# Autodesk Inventor assembly: ForeArm
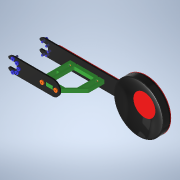
[picture p0: Inventor's stored thumbnail of the model, 180x180]
Saved by Autodesk Inventor 2020 (Build 240168000, 168)
## iProperties
Created: 2022-01-10
Part Number: ForeArm
Document SubType Name: Assembly
Designer: Masato Kubotera
Author: Masato Kubotera
## Documents named in this file (12)
- C:\Users\MasatoKubotera\Documents\Inventor\OpenPlatform_ver3_0 - prototype\UpperBody\Arm\ForeArm.iam
- C:\Users\MasatoKubotera\Documents\Inventor\OpenPlatform_ver3_0 - prototype\UpperBody\Arm\ForeArm_outside_frame.ipt
- C:\Users\MasatoKubotera\Documents\Inventor\OpenPlatform_ver3_0 - prototype\UpperBody\Arm\ForeArm_hand.ipt
- C:\Users\MasatoKubotera\Documents\Inventor\OpenPlatform_ver3_0 - prototype\UpperBody\Arm\ForeArm_inside_frame.ipt
- C:\Users\MasatoKubotera\Documents\Inventor\OpenPlatform_ver3_0 - prototype\ReadyMade\InsertNut\UD-43040.ipt
- C:\Users\MasatoKubotera\Documents\Inventor\OpenPlatform_ver3_0 - prototype\ReadyMade\Screw\M3-6.ipt
- C:\Users\MasatoKubotera\Documents\Inventor\OpenPlatform_ver3_0 - prototype\ReadyMade\Screw\M2_6-6.ipt
- C:\Users\MasatoKubotera\Documents\Inventor\OpenPlatform_ver3_0 - prototype\ReadyMade\InsertNut\IRU-304SW.ipt
- C:\Users\MasatoKubotera\Documents\Inventor\OpenPlatform_ver3_0 - prototype\UpperBody\Arm\ForeArm_diagonal.ipt
- C:\Users\MasatoKubotera\Documents\Inventor\OpenPlatform_ver3_0 - prototype\UpperBody\Arm\ForeArm_outside_cloth.ipt
- C:\Users\MasatoKubotera\Documents\Inventor\OpenPlatform_ver3_0 - prototype\ReadyMade\Bush\L3040-8110TB.ipt
- C:\Users\MasatoKubotera\Documents\Inventor\OpenPlatform_ver3_0 - prototype\ReadyMade\Screw\M3-8.ipt
## Components (34 placed, 11 different names)
1. ForeArm_outside_frame:1 — 挿入:7, 挿入:9, 挿入:10, 挿入:16, 挿入:17, 挿入:23, 挿入:24, 挿入:28, 挿入:31, 挿入:32, 挿入:33, 挿入:34, メイト:1, メイト:2, フラッシュ:1, 挿入:8, 挿入:39, 挿入:41, 挿入:42, 挿入:43
2. ForeArm_hand:1 — 挿入:1, 挿入:2, 挿入:3, 挿入:4, 挿入:8
3. ForeArm_inside_frame:1 — 挿入:25, 挿入:26, 挿入:29, 挿入:30, 挿入:35, 挿入:36, 挿入:37, 挿入:38, 挿入:40
4. ForeArm_diagonal:1 — 挿入:19, 挿入:20, 挿入:21, 挿入:22
5. M2_6-6:9 — 挿入:39
6. M2_6-6:10 — 挿入:40
7. ForeArm_outside_cloth:1 — 挿入:47, 挿入:48, 挿入:49
8. L3040-8110TB:1 — 挿入:41, 挿入:47, 挿入:50
9. L3040-8110TB:2 — 挿入:42, 挿入:48, 挿入:51
10. L3040-8110TB:3 — 挿入:43, 挿入:46, 挿入:49
11. M3-8:2 — 挿入:50
12. M3-8:3 — 挿入:51
13. M3-6:10 — 挿入:30
14. M3-6:9 — 挿入:29
15. M3-6:8 — 挿入:28
16. M2_6-6:8 — 挿入:38
17. M2_6-6:7 — 挿入:37
18. M2_6-6:6 — 挿入:36
19. M2_6-6:5 — 挿入:35
20. M2_6-6:4 — 挿入:34
21. M2_6-6:3 — 挿入:33
22. M2_6-6:2 — 挿入:32
23. M2_6-6:1 — 挿入:31
24. M3-6:5 — 挿入:17
25. M3-6:4 — 挿入:16
26. M3-8:1 — 挿入:46
27. UD-43040:4 — 挿入:4, 挿入:10
28. UD-43040:3 — 挿入:3, 挿入:9
29. UD-43040:2 — 挿入:2
30. UD-43040:1 — 挿入:1, 挿入:7
31. IRU-304SW:1 — 挿入:19, 挿入:23
32. IRU-304SW:2 — 挿入:20, 挿入:24
33. IRU-304SW:3 — 挿入:21, 挿入:25
34. IRU-304SW:4 — 挿入:22, 挿入:26
## Relationships (43: Insert 40, Mate 2, Flush 1)
- 挿入:1 [Insert]: ForeArm_hand:1 ↔ UD-43040:1
- 挿入:2 [Insert]: ForeArm_hand:1 ↔ UD-43040:2
- 挿入:3 [Insert]: ForeArm_hand:1 ↔ UD-43040:3
- 挿入:4 [Insert]: ForeArm_hand:1 ↔ UD-43040:4
- 挿入:7 [Insert]: ForeArm_outside_frame:1 ↔ UD-43040:1
- 挿入:8 [Insert]: ForeArm_outside_frame:1 ↔ ForeArm_hand:1
- 挿入:9 [Insert]: ForeArm_outside_frame:1 ↔ UD-43040:3
- 挿入:10 [Insert]: ForeArm_outside_frame:1 ↔ UD-43040:4
- 挿入:16 [Insert]: ForeArm_outside_frame:1 ↔ M3-6:4
- 挿入:17 [Insert]: ForeArm_outside_frame:1 ↔ M3-6:5
- 挿入:19 [Insert]: ForeArm_diagonal:1 ↔ IRU-304SW:1
- 挿入:20 [Insert]: ForeArm_diagonal:1 ↔ IRU-304SW:2
- 挿入:21 [Insert]: ForeArm_diagonal:1 ↔ IRU-304SW:3
- 挿入:22 [Insert]: ForeArm_diagonal:1 ↔ IRU-304SW:4
- 挿入:23 [Insert]: ForeArm_outside_frame:1 ↔ IRU-304SW:1
- 挿入:24 [Insert]: ForeArm_outside_frame:1 ↔ IRU-304SW:2
- 挿入:25 [Insert]: ForeArm_inside_frame:1 ↔ IRU-304SW:3
- 挿入:26 [Insert]: ForeArm_inside_frame:1 ↔ IRU-304SW:4
- 挿入:28 [Insert]: ForeArm_outside_frame:1 ↔ M3-6:8
- 挿入:29 [Insert]: ForeArm_inside_frame:1 ↔ M3-6:9
- 挿入:30 [Insert]: ForeArm_inside_frame:1 ↔ M3-6:10
- 挿入:31 [Insert]: ForeArm_outside_frame:1 ↔ M2_6-6:1
- 挿入:32 [Insert]: ForeArm_outside_frame:1 ↔ M2_6-6:2
- 挿入:33 [Insert]: ForeArm_outside_frame:1 ↔ M2_6-6:3
- 挿入:34 [Insert]: ForeArm_outside_frame:1 ↔ M2_6-6:4
- 挿入:35 [Insert]: ForeArm_inside_frame:1 ↔ M2_6-6:5
- 挿入:36 [Insert]: ForeArm_inside_frame:1 ↔ M2_6-6:6
- 挿入:37 [Insert]: ForeArm_inside_frame:1 ↔ M2_6-6:7
- 挿入:38 [Insert]: ForeArm_inside_frame:1 ↔ M2_6-6:8
- メイト:1 [Mate]: ForeArm_outside_frame:1
- メイト:2 [Mate]: ForeArm_outside_frame:1
- フラッシュ:1 [Flush]: ForeArm_outside_frame:1
- 挿入:39 [Insert]: ForeArm_outside_frame:1 ↔ M2_6-6:9
- 挿入:40 [Insert]: ForeArm_inside_frame:1 ↔ M2_6-6:10
- 挿入:41 [Insert]: ForeArm_outside_frame:1 ↔ L3040-8110TB:1
- 挿入:42 [Insert]: ForeArm_outside_frame:1 ↔ L3040-8110TB:2
- 挿入:43 [Insert]: ForeArm_outside_frame:1 ↔ L3040-8110TB:3
- 挿入:46 [Insert]: L3040-8110TB:3 ↔ M3-8:1
- 挿入:47 [Insert]: ForeArm_outside_cloth:1 ↔ L3040-8110TB:1
- 挿入:48 [Insert]: ForeArm_outside_cloth:1 ↔ L3040-8110TB:2
- 挿入:49 [Insert]: ForeArm_outside_cloth:1 ↔ L3040-8110TB:3
- 挿入:50 [Insert]: L3040-8110TB:1 ↔ M3-8:2
- 挿入:51 [Insert]: L3040-8110TB:2 ↔ M3-8:3
